# Autodesk Inventor assembly: gears
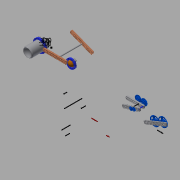
[picture p0: Inventor's stored thumbnail of the model, 180x180]
Saved by Autodesk Inventor 2019.3 (Build 233278000, 278)
## iProperties
Created: 2019-01-24
Part Number: gears
Document SubType Name: Assembly
Designer: Varga Daniel
Author: Varga Daniel
## Documents named in this file (28)
- C:\!_Dani\!_cloud\OneDrive\!_munka\Revolution\RevvyDemoKit\Structural parts\Part_test_Assembly.iam
- C:\!_Dani\!_cloud\OneDrive\!_munka\Revolution\RevvyDemoKit\Structural parts\Beams\Straight Beams\S2+x2\S16x2.iam
- C:\!_Dani\!_cloud\OneDrive\!_munka\Revolution\RevvyDemoKit\Structural parts\Beams\Straight Beams\S2+x2.iam
- C:\!_Dani\!_cloud\OneDrive\!_munka\Revolution\RevvyDemoKit\Structural parts\Beams\Curved beams\CB4H.ipt
- C:\!_Dani\!_cloud\OneDrive\!_munka\Revolution\RevvyDemoKit\Structural parts\Beams\Curved beams\CB6H.ipt
- C:\!_Dani\!_cloud\OneDrive\!_munka\Revolution\RevvyDemoKit\Structural parts\Beams\Curved beams\cocacola can.ipt
- C:\!_Dani\!_cloud\OneDrive\!_munka\Revolution\RevvyDemoKit\Structural parts\Beams\Straight Beams\S2+x1\S2x1.iam
- C:\!_Dani\!_cloud\OneDrive\!_munka\Revolution\RevvyDemoKit\Structural parts\Beams\Straight Beams\S2+x1.iam
- C:\!_Dani\!_cloud\OneDrive\!_munka\Revolution\RevvyDemoKit\Structural parts\Beams\Curved beams\Table tennis ball.ipt
- C:\!_Dani\!_cloud\OneDrive\!_munka\Revolution\RevvyDemoKit\Structural parts\Beams\Round Beams\RB1+\RB16.iam
- C:\!_Dani\!_cloud\OneDrive\!_munka\Revolution\RevvyDemoKit\Structural parts\Beams\Round Beams\RB1+.iam
- C:\!_Dani\!_cloud\OneDrive\!_munka\Revolution\RevvyDemoKit\Structural parts\Axles\AXp2+c\AXp2c.ipt
- C:\!_Dani\!_cloud\OneDrive\!_munka\Revolution\RevvyDemoKit\Structural parts\Axles\AXp2+c.ipt
- C:\!_Dani\!_cloud\OneDrive\!_munka\Revolution\RevvyDemoKit\Structural parts\Axles\AXp2+c\AXp3c.ipt
- C:\!_Dani\!_cloud\OneDrive\!_munka\Revolution\RevvyDemoKit\Structural parts\Axles\AXp2+s\AXp12s.ipt
- C:\!_Dani\!_cloud\OneDrive\!_munka\Revolution\RevvyDemoKit\Structural parts\Axles\AXp2+s.ipt
- C:\!_Dani\!_cloud\OneDrive\!_munka\Revolution\RevvyDemoKit\Structural parts\Axles\AXp2+s\AXp6s.ipt
- C:\!_Dani\!_cloud\OneDrive\!_munka\Revolution\RevvyDemoKit\Structural parts\Axles\AXp2+s\AXp3s.ipt
- C:\!_Dani\!_cloud\OneDrive\!_munka\Revolution\RevvyDemoKit\Structural parts\Connetor Pins\CP1+x1+\CP2x2.iam
- C:\!_Dani\!_cloud\OneDrive\!_munka\Revolution\RevvyDemoKit\Structural parts\Connetor Pins\CP1+x1+.iam
- C:\!_Dani\!_cloud\OneDrive\!_munka\Revolution\RevvyDemoKit\Structural parts\Connetor Pins\CP1+x1+\CP1x1.iam
- C:\!_Dani\!_cloud\OneDrive\!_munka\Revolution\RevvyDemoKit\Structural parts\Gears\G40.iam
- C:\!_Dani\!_cloud\OneDrive\!_munka\Revolution\RevvyDemoKit\Structural parts\Beams\Round Beams\RB1+\RB2.iam
- C:\!_Dani\!_cloud\OneDrive\!_munka\Revolution\RevvyDemoKit\Structural parts\Gears\G20.iam
- C:\!_Dani\!_cloud\OneDrive\!_munka\Revolution\RevvyDemoKit\Structural parts\Axles\AXp3+p\AXp4p.iam
- C:\!_Dani\!_cloud\OneDrive\!_munka\Revolution\RevvyDemoKit\Structural parts\Axles\AXp3+p.iam
- C:\!_Dani\!_cloud\OneDrive\!_munka\Revolution\RevvyDemoKit\Structural parts\Beams\Straight Beams\S2+x2\S12x2.iam
- C:\!_Dani\!_cloud\OneDrive\!_munka\Revolution\RevvyDemoKit\Structural parts\Gears\G60.iam
## Components (34 placed, 20 different names)
1. S16x2:1 [sub-assembly] — Mate:1, Mate:2, Mate:3, Mate:4, Mate:14, Mate:15, Mate:16, Mate:17, Mate:25, Mate:26, Mate:29, Mate:30
2. S16x2:2 [sub-assembly] — Mate:31, Mate:32
3. CB4H:1 — Mate:14, Mate:15, Mate:19, Mate:26, Tangent:1
4. CB6H:1 — Mate:1, Mate:2, Mate:6, Mate:12, Mate:13
5. cocacola can:1 — Mate:5, Flush:1, Mate:6, Mate:11
6. CB6H:2 — Mate:3, Mate:4, Mate:5, Flush:1, Mate:9, Mate:10
7. S2x1:1 [sub-assembly] — Mate:7, Mate:8, Mate:9, Mate:10
8. S2x1:2 [sub-assembly] — Mate:12, Mate:13, Tangent:2
9. S2x1:3 [sub-assembly] — Mate:22, Mate:23, Mate:24
10. CB6H:3 — Mate:7, Mate:8, Mate:11, Tangent:2
11. Table tennis ball:1 — Mate:18, Mate:19, Mate:20, Mate:21
12. CB4H:2 — Mate:16, Mate:17, Mate:18, Mate:21, Flush:2, Mate:22, Mate:23, Mate:25
13. CB4H:3 — Mate:20, Flush:2, Mate:24, Mate:27, Mate:28
14. S2x1:4 [sub-assembly] — Mate:27, Mate:28, Tangent:1
15. RB16:1 [sub-assembly] — Mate:29, Mate:30, Mate:31, Mate:32
16. AXp2c:2
17. AXp3c:3
18. AXp12s:1
19. AXp6s:2
20. AXp3s:3
21. CP2x2:1 [sub-assembly]
22. CP1x1:3 [sub-assembly]
23. S16x2:5 [sub-assembly] — Mate:64, Mate:65, Mate:66, Mate:67, Mate:68, Mate:69
24. G40:1 [sub-assembly] — Flush:3, Angle:4, Mate:57, Mate:58
25. S12x2:6 [sub-assembly] — Mate:43, Mate:44, Mate:50, Mate:51, Mate:55, Mate:56, Mate:57, Mate:58
26. RB2:2 [sub-assembly] — Mate:43, Mate:44, Mate:45, Mate:52
27. S12x2:7 [sub-assembly] — Mate:45, Mate:52, Mate:53, Mate:59, Mate:60, Angle:6
28. G40:2 [sub-assembly] — Mate:46, Angle:2, Mate:47, Mate:49, Flush:3, Angle:4, Mate:55, Mate:56
29. G20:1 [sub-assembly] — Mate:48, Mate:49, Angle:3, Mate:53, Mate:59, Flush:4, Angle:5
30. AXp4p:1 [sub-assembly]
31. AXp4p:2 [sub-assembly] — Mate:46, Angle:2, Mate:47, Mate:48, Angle:3, Mate:50, Mate:51
32. G20:2 [sub-assembly] — Mate:60, Flush:4, Angle:5, Angle:6
33. G60:1 [sub-assembly] — Mate:67, Mate:68, Mate:69
34. G60:2 [sub-assembly] — Mate:64, Mate:65, Mate:66
## Relationships (66: Mate 55, Angle 5, Flush 4, Tangent 2)
- Mate:1: S16x2:1 ↔ CB6H:1
- Mate:2: S16x2:1 ↔ CB6H:1
- Mate:3: S16x2:1 ↔ CB6H:2
- Mate:4: S16x2:1 ↔ CB6H:2
- Mate:5: cocacola can:1 ↔ CB6H:2
- Flush:1 (-30 mm): cocacola can:1 ↔ CB6H:2
- Mate:6: CB6H:1 ↔ cocacola can:1
- Mate:7: S2x1:1 ↔ CB6H:3
- Mate:8: S2x1:1 ↔ CB6H:3
- Mate:9: CB6H:2 ↔ S2x1:1
- Mate:10: CB6H:2 ↔ S2x1:1
- Mate:11: cocacola can:1 ↔ CB6H:3
- Mate:12: CB6H:1 ↔ S2x1:2
- Mate:13: CB6H:1 ↔ S2x1:2
- Mate:14: S16x2:1 ↔ CB4H:1
- Mate:15: S16x2:1 ↔ CB4H:1
- Mate:16: S16x2:1 ↔ CB4H:2
- Mate:17: S16x2:1 ↔ CB4H:2
- Mate:18: Table tennis ball:1 ↔ CB4H:2
- Mate:19: CB4H:1 ↔ Table tennis ball:1
- Mate:20: Table tennis ball:1 ↔ CB4H:3
- Mate:21: Table tennis ball:1 ↔ CB4H:2
- Flush:2: CB4H:2 ↔ CB4H:3
- Mate:22: S2x1:3 ↔ CB4H:2
- Mate:23: S2x1:3 ↔ CB4H:2
- Mate:24: S2x1:3 ↔ CB4H:3
- Mate:25: S16x2:1 ↔ CB4H:2
- Mate:26: S16x2:1 ↔ CB4H:1
- Mate:27: CB4H:3 ↔ S2x1:4
- Mate:28: CB4H:3 ↔ S2x1:4
- Tangent:1: CB4H:1 ↔ S2x1:4
- Tangent:2: S2x1:2 ↔ CB6H:3
- Mate:29: S16x2:1 ↔ RB16:1
- Mate:30: S16x2:1 ↔ RB16:1
- Mate:31: S16x2:2 ↔ RB16:1
- Mate:32: S16x2:2 ↔ RB16:1
- Mate:43: S12x2:6 ↔ RB2:2
- Mate:44: S12x2:6 ↔ RB2:2
- Mate:45: RB2:2 ↔ S12x2:7
- Mate:46: G40:2 ↔ AXp4p:2
- Angle:2 (0 deg): G40:2 ↔ AXp4p:2
- Mate:47: G40:2 ↔ AXp4p:2
- Mate:48: G20:1 ↔ AXp4p:2
- Mate:49: G40:2 ↔ G20:1
- Angle:3 (0 deg): G20:1 ↔ AXp4p:2
- Mate:50: S12x2:6 ↔ AXp4p:2
- Mate:51: S12x2:6 ↔ AXp4p:2
- Mate:52: RB2:2 ↔ S12x2:7
- Mate:53: S12x2:7 ↔ G20:1
- Flush:3: G40:1 ↔ G40:2
- Angle:4 (0 deg): G40:1 ↔ G40:2
- Mate:55: S12x2:6 ↔ G40:2
- Mate:56: S12x2:6 ↔ G40:2
- Mate:57: G40:1 ↔ S12x2:6
- Mate:58: G40:1 ↔ S12x2:6
- Mate:59: S12x2:7 ↔ G20:1
- Mate:60: S12x2:7 ↔ G20:2
- Flush:4: G20:1 ↔ G20:2
- Angle:5 (0 deg): G20:1 ↔ G20:2
- Angle:6 (0 deg): S12x2:7 ↔ G20:2
- Mate:64: S16x2:5 ↔ G60:2
- Mate:65: S16x2:5 ↔ G60:2
- Mate:66: S16x2:5 ↔ G60:2
- Mate:67: S16x2:5 ↔ G60:1
- Mate:68: S16x2:5 ↔ G60:1
- Mate:69: S16x2:5 ↔ G60:1
